# Autodesk Inventor assembly: invacare assy
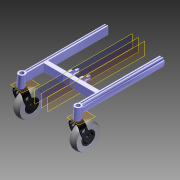
[picture p0: Inventor's stored thumbnail of the model, 180x180]
Saved by Autodesk Inventor 2012 (Build 160160000, 160)
## iProperties
Created: 2012-03-07
Part Number: invacare assy
Document SubType Name: Assembly
Designer: esv
Author: esv
## Documents named in this file (3)
- C:\Users\esv\masters\CAD\Invacare\invacare assy.iam
- C:\Users\esv\masters\CAD\Invacare\caster assy.iam
- C:\Users\esv\masters\CAD\Invacare\frame.ipt
## Components (3 placed, 2 different names)
1. caster assy:1 [sub-assembly] — Insert:1
2. caster assy:2 [sub-assembly] — Insert:2
3. frame:1 — Insert:1, Insert:2
## Relationships (2: Insert 2)
- Insert:1: caster assy:1 ↔ frame:1
- Insert:2: caster assy:2 ↔ frame:1
